# Autodesk Inventor assembly: Transmisión de correa trapezoidal
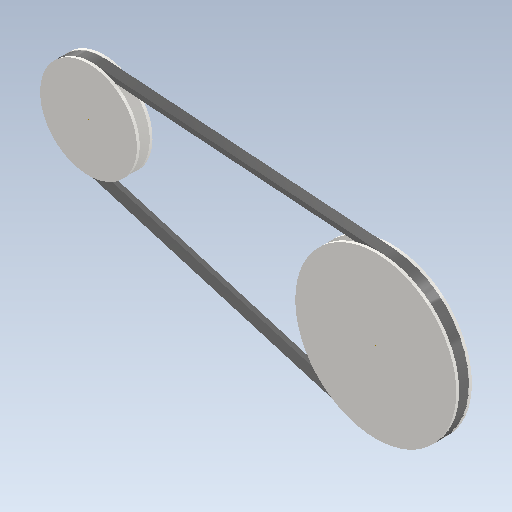
[picture p0: Inventor's stored thumbnail of the model, 512x512]
Saved by Autodesk Inventor 2020 (Build 240168000, 168)
## iProperties
ClientObjectVersion: 1
Created: 2020-12-08
Part Number: Transmisión de correa trapezoidal
Document SubType Name: Assembly
Designer: DanielAlvaradoPelaez
Author: DanielAlvaradoPelaez
## Documents named in this file (4)
- C:\Users\DanielAlvaradoPelaez\Desktop\Espol S5\diseño y simulacion de maquinas\deber\tarea 4\ac-motor-14.snapshot.1\Assembly1\Design Accelerator\Transmisión de correa trapezoidal1.iam
- C:\Users\DanielAlvaradoPelaez\Desktop\Espol S5\diseño y simulacion de maquinas\deber\tarea 4\ac-motor-14.snapshot.1\Assembly1\Design Accelerator\Correa trapezoidal1.ipt
- C:\Users\DanielAlvaradoPelaez\Desktop\Espol S5\diseño y simulacion de maquinas\deber\tarea 4\ac-motor-14.snapshot.1\Assembly1\Design Accelerator\Polea ranurada11.ipt
- C:\Users\DanielAlvaradoPelaez\Desktop\Espol S5\diseño y simulacion de maquinas\deber\tarea 4\ac-motor-14.snapshot.1\Assembly1\Design Accelerator\Polea ranurada21.ipt
## Components (3 placed, 3 different names)
1. Polea ranurada1:1 — Nivelación:1, Coincidencia:1, Rotación:1
2. Polea ranurada2:1 — Nivelación:2, Coincidencia:2, Rotación:1
3. Correa trapezoidal:1 — Nivelación:1, Coincidencia:1, Nivelación:2, Coincidencia:2
## Component patterns: (1 elements, first: Correa trapezoidal:1)
## Relationships (5: Flush 2, Mate 2, RelateRotation 1)
- Nivelación:1 [Flush]: Polea ranurada1:1 ↔ Correa trapezoidal:1
- Coincidencia:1 [Mate]: Polea ranurada1:1 ↔ Correa trapezoidal:1
- Nivelación:2 [Flush]: Polea ranurada2:1 ↔ Correa trapezoidal:1
- Coincidencia:2 [Mate]: Polea ranurada2:1 ↔ Correa trapezoidal:1
- Rotación:1 [RelateRotation] (1.6949 ul): Polea ranurada1:1 ↔ Polea ranurada2:1
